# Autodesk Inventor assembly: outer_MIR
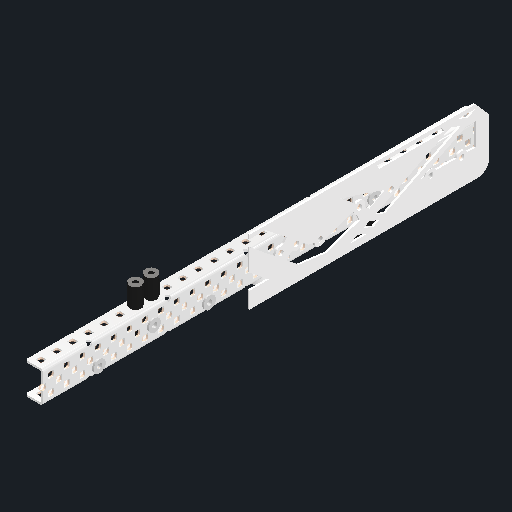
[picture p0: Inventor's stored thumbnail of the model, 512x512]
Saved by Autodesk Inventor 2024 (Build 280153000, 153)
## iProperties
Created: 2023-10-29
Part Number: outer_MIR
Document SubType Name: Assembly
Designer: avere
Author: Averey Ku
## Documents named in this file (15)
- C:\Users\avere\Documents\rbp_cad\zoomba_v0.2\chassis\mirrored_parts\outer_MIR.iam
- C:\Users\avere\Documents\rbp_cad\zoomba_v0.2\chassis\mirrored_parts\Insert Circle_MIR.ipt
- C:\Users\avere\Documents\rbp_cad\zoomba_v0.2\chassis\mirrored_parts\Alu C 1x2x1x28_MIR.ipt
- C:\Users\avere\Documents\rbp_cad\zoomba_v0.2\chassis\mirrored_parts\.375 OD Aluminum Spacer 0.875_MIR.ipt
- C:\Users\avere\Documents\rbp_cad\VEX-CAD-Inventor-1.41\Structure\Standoff\Standoff .875.ipt
- C:\Users\avere\Documents\rbp_cad\VEX-CAD-Inventor-1.41\Structure\Standoff.ipt
- C:\Users\avere\Documents\rbp_cad\zoomba_v0.2\chassis\drivebay\custom_parts\washer_thick.ipt
- C:\Users\avere\Documents\rbp_cad\VEX-CAD-Inventor-1.41\Motion\Spacers\Spacer Nylon .500 OD\NSpacer White .500 OD x .250.ipt
- C:\Users\avere\Documents\rbp_cad\VEX-CAD-Inventor-1.41\Motion\Spacers\Spacer Nylon .500 OD.ipt
- C:\Users\avere\Documents\rbp_cad\zoomba_v0.2\chassis\drivebay\custom_parts\sideplate.ipt
- C:\Users\avere\Documents\rbp_cad\VEX-CAD-Inventor-1.41\Motion\Spacers\Spacer Nylon .375 OD\NSpacer .375 OD x .500.ipt
- C:\Users\avere\Documents\rbp_cad\VEX-CAD-Inventor-1.41\Motion\Spacers\Spacer Nylon .375 OD.ipt
- C:\Users\avere\Documents\rbp_cad\VEX-CAD-Inventor-1.41\Motion\Spacers\Spacer Nylon .375 OD\NSpacer .375 OD x .125.ipt
- C:\Users\avere\Documents\rbp_cad\VEX-CAD-Inventor-1.41\Motion\Spacers\Washer Steel\SWasher .375 OD x .031250.ipt
- C:\Users\avere\Documents\rbp_cad\VEX-CAD-Inventor-1.41\Motion\Spacers\Washer Steel.ipt
## Components (27 placed, 10 different names)
1. Insert Circle_MIR:1 — Insert:1
2. Insert Circle_MIR:2 — Insert:2
3. Insert Circle_MIR:3 — Insert:3
4. Insert Circle_MIR:4 — Insert:4
5. Insert Circle_MIR:5 — Insert:5
6. Insert Circle_MIR:6 — Insert:6
7. Insert Circle_MIR:7 — Insert:7
8. Alu C 1x2x1x28_MIR:1 — Insert:7, Insert:6, Insert:5, Insert:4, Insert:3, Insert:2, Insert:1, Insert:8, Insert:17, Insert:19, Insert:20, Insert:22, Insert:23, Mate:1, Insert:34, Insert:35, Insert:36, Insert:41
9. .375 OD Aluminum Spacer 0.875_MIR:1 — Insert:8
10. Standoff .875:1 — Insert:17
11. Standoff .875:3 — Insert:19
12. Standoff .875:4 — Insert:20
13. washer_thick:1 — Insert:22
14. NSpacer White .500 OD x .250:1
15. sideplate:1 — Insert:23, Mate:1
16. NSpacer .375 OD x .500:5 — Insert:35
17. NSpacer .375 OD x .125:6
18. SWasher .375 OD x .031250:3
19. NSpacer .375 OD x .500:7 — Insert:34
20. NSpacer .375 OD x .125:8
21. SWasher .375 OD x .031250:4
22. NSpacer .375 OD x .125:9 — Insert:37, Insert:38
23. SWasher .375 OD x .031250:5 — Insert:38
24. NSpacer .375 OD x .500:10 — Insert:36, Insert:37
25. NSpacer .375 OD x .125:11
26. SWasher .375 OD x .031250:6
27. NSpacer .375 OD x .500:12 — Insert:41
## Relationships (27: Insert 26, Mate 1)
- Insert:7: Insert Circle_MIR:7 ↔ Alu C 1x2x1x28_MIR:1
- Insert:6: Insert Circle_MIR:6 ↔ Alu C 1x2x1x28_MIR:1
- Insert:5: Insert Circle_MIR:5 ↔ Alu C 1x2x1x28_MIR:1
- Insert:4: Insert Circle_MIR:4 ↔ Alu C 1x2x1x28_MIR:1
- Insert:3: Insert Circle_MIR:3 ↔ Alu C 1x2x1x28_MIR:1
- Insert:2: Insert Circle_MIR:2 ↔ Alu C 1x2x1x28_MIR:1
- Insert:1: Insert Circle_MIR:1 ↔ Alu C 1x2x1x28_MIR:1
- Insert:8: Alu C 1x2x1x28_MIR:1 ↔ .375 OD Aluminum Spacer 0.875_MIR:1
- Insert:17: Alu C 1x2x1x28_MIR:1 ↔ Standoff .875:1
- Insert:19: Alu C 1x2x1x28_MIR:1 ↔ Standoff .875:3
- Insert:20: Alu C 1x2x1x28_MIR:1 ↔ Standoff .875:4
- [Insert]: washer_thick:1 ↔ NSpacer White .500 OD x .250:1
- Insert:22: Alu C 1x2x1x28_MIR:1 ↔ washer_thick:1
- Insert:23: Alu C 1x2x1x28_MIR:1 ↔ sideplate:1
- Mate:1: Alu C 1x2x1x28_MIR:1 ↔ sideplate:1
- [Insert]: NSpacer .375 OD x .500:5 ↔ NSpacer .375 OD x .125:6
- [Insert]: NSpacer .375 OD x .125:6 ↔ SWasher .375 OD x .031250:3
- [Insert]: NSpacer .375 OD x .500:7 ↔ NSpacer .375 OD x .125:8
- [Insert]: NSpacer .375 OD x .125:8 ↔ SWasher .375 OD x .031250:4
- Insert:34: Alu C 1x2x1x28_MIR:1 ↔ NSpacer .375 OD x .500:7
- Insert:35: Alu C 1x2x1x28_MIR:1 ↔ NSpacer .375 OD x .500:5
- Insert:36: Alu C 1x2x1x28_MIR:1 ↔ NSpacer .375 OD x .500:10
- Insert:37: NSpacer .375 OD x .125:9 ↔ NSpacer .375 OD x .500:10
- Insert:38: NSpacer .375 OD x .125:9 ↔ SWasher .375 OD x .031250:5
- [Insert]: NSpacer .375 OD x .125:11 ↔ NSpacer .375 OD x .500:12
- [Insert]: NSpacer .375 OD x .125:11 ↔ SWasher .375 OD x .031250:6
- Insert:41: Alu C 1x2x1x28_MIR:1 ↔ NSpacer .375 OD x .500:12
## Named parameters: d30_d25 = 0 mm, d31_d26 = 0 mm, d32_d25 = 0 mm, d33_d26 = 0 mm, d39_d37 = 0 mm, d40_d38 = 0 mm
